# Autodesk Inventor assembly: towerbottom2.2
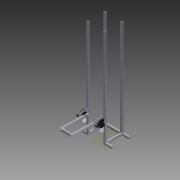
[picture p0: Inventor's stored thumbnail of the model, 180x180]
Saved by Autodesk Inventor 2011 SP1 (Build 150282100, 282)
## iProperties
Created: 2012-01-19
Part Number: towerbottom2.2
Document SubType Name: Assembly
Designer: Christopher
Author: Christopher
## Documents named in this file (12)
- C:\Users\Christopher\Documents\Christopher\FIRST\Inventor files\2012\tower bottom second design\towerbottom2.2.iam
- C:\Users\Christopher\Documents\Christopher\FIRST\Inventor files\2012\tower first design\towertallbackthing.ipt
- C:\Users\Christopher\Documents\Christopher\FIRST\Inventor files\2012\tower bottom second design\tower horizontal brace 17.5in.ipt
- C:\Users\Christopher\Documents\Christopher\FIRST\Inventor files\2012\tower bottom second design\towermiddle8inbrace.ipt
- C:\Users\Christopher\Documents\Christopher\FIRST\Inventor files\2012\tower bottom second design\towerside4.5inbrace.ipt
- C:\Users\Christopher\Documents\Christopher\FIRST\Inventor files\2011\Kit of Parts\motors\Motors_Denso_262100-3030.ipt
- C:\Users\Christopher\Documents\Christopher\FIRST\Inventor files\2011\Kit of Parts\motors\Motors_Denso_262100-3040.ipt
- C:\Users\Christopher\Documents\Christopher\FIRST\Inventor files\2012\tower bottom second design\window motor plate.ipt
- C:\Users\Christopher\Documents\Christopher\FIRST\Inventor files\2012\tower bottom second design\ramp1.ipt
- C:\Users\Christopher\Documents\Christopher\FIRST\Inventor files\2011\Kit of Parts\motors\Motors_Pelham Plastics_Denso-6.ipt
- C:\Users\Christopher\Documents\Christopher\FIRST\Inventor files\2012\tower bottom second design\bambar 12 in.ipt
- C:\Users\Christopher\Documents\Christopher\FIRST\Inventor files\2012\tower bottom second design\bambar 8.5 inch.ipt
## Components (19 placed, 11 different names)
1. towertallbackthing:1 — Mate:10, Flush:17, Flush:18, Flush:20, Mate:22
2. towertallbackthing:2 — Mate:9, Flush:21, Flush:22, Mate:21, Flush:27
3. towertallbackthing:3 — Mate:5, Flush:8, Flush:9
4. towertallbackthing:4 — Mate:6, Flush:10, Flush:11
5. tower horizontal brace 17.5in:2 — Mate:2, Flush:3, Flush:4, Mate:5, Flush:8, Flush:9, Mate:6, Flush:10, Flush:11, Flush:12, Mate:7, Flush:13, Mate:12, Flush:19
6. towermiddle8inbrace:1 — Mate:2, Flush:3, Flush:4, Mate:11, Flush:15, Flush:16, Flush:18, Mate:13
7. towermiddle8inbrace:2 — Flush:12, Mate:7, Flush:13, Mate:8, Flush:14, Mate:18, Flush:27
8. towerside4.5inbrace:1 — Mate:10, Mate:11, Flush:15, Flush:16, Flush:17, Mate:15
9. towerside4.5inbrace:2 — Mate:8, Flush:14, Mate:9, Mate:17, Flush:22
10. Motors_Denso_262100-3030:1 — Insert:1, Insert:4
11. Motors_Denso_262100-3040:1 — Insert:2, Insert:3
12. window motor plate:1 — Insert:1, Mate:15, Flush:20, Mate:22
13. window motor plate:2 — Mate:17, Flush:21, Insert:2, Mate:18, Mate:21
14. ramp1:1 — Mate:12, Flush:19, Mate:13
15. Motors_Pelham Plastics_Denso-6:1 — Insert:3, Insert:5, Insert:6
16. Motors_Pelham Plastics_Denso-6:2 — Insert:4
17. bambar 12 in:1 — Flush:23, Mate:19, Flush:24
18. bambar 12 in:2 — Mate:20, Flush:25, Flush:26, Insert:5, Insert:6
19. bambar 8.5 inch:1 — Flush:23, Mate:19, Flush:24, Mate:20, Flush:25, Flush:26
## Relationships (45: Flush 22, Mate 17, Insert 6)
- Mate:2: tower horizontal brace 17.5in:2 ↔ towermiddle8inbrace:1
- Flush:3: tower horizontal brace 17.5in:2 ↔ towermiddle8inbrace:1
- Flush:4 (-88.9 mm): tower horizontal brace 17.5in:2 ↔ towermiddle8inbrace:1
- Mate:5: towertallbackthing:3 ↔ tower horizontal brace 17.5in:2
- Flush:8: towertallbackthing:3 ↔ tower horizontal brace 17.5in:2
- Flush:9 (88.9 mm): towertallbackthing:3 ↔ tower horizontal brace 17.5in:2
- Mate:6: towertallbackthing:4 ↔ tower horizontal brace 17.5in:2
- Flush:10: towertallbackthing:4 ↔ tower horizontal brace 17.5in:2
- Flush:11 (88.9 mm): towertallbackthing:4 ↔ tower horizontal brace 17.5in:2
- Flush:12: tower horizontal brace 17.5in:2 ↔ towermiddle8inbrace:2
- Mate:7: tower horizontal brace 17.5in:2 ↔ towermiddle8inbrace:2
- Flush:13 (-88.9 mm): tower horizontal brace 17.5in:2 ↔ towermiddle8inbrace:2
- Mate:8: towermiddle8inbrace:2 ↔ towerside4.5inbrace:2
- Flush:14: towermiddle8inbrace:2 ↔ towerside4.5inbrace:2
- Mate:9: towertallbackthing:2 ↔ towerside4.5inbrace:2
- Mate:10: towertallbackthing:1 ↔ towerside4.5inbrace:1
- Mate:11: towermiddle8inbrace:1 ↔ towerside4.5inbrace:1
- Flush:15: towermiddle8inbrace:1 ↔ towerside4.5inbrace:1
- Flush:16: towermiddle8inbrace:1 ↔ towerside4.5inbrace:1
- Flush:17: towertallbackthing:1 ↔ towerside4.5inbrace:1
- Flush:18: towertallbackthing:1 ↔ towermiddle8inbrace:1
- Insert:1: Motors_Denso_262100-3030:1 ↔ window motor plate:1
- Mate:12: tower horizontal brace 17.5in:2 ↔ ramp1:1
- Flush:19: tower horizontal brace 17.5in:2 ↔ ramp1:1
- Mate:13: towermiddle8inbrace:1 ↔ ramp1:1
- Mate:15 (203.2 mm): towerside4.5inbrace:1 ↔ window motor plate:1
- Flush:20: towertallbackthing:1 ↔ window motor plate:1
- Mate:17 (203.2 mm): towerside4.5inbrace:2 ↔ window motor plate:2
- Flush:21: towertallbackthing:2 ↔ window motor plate:2
- Flush:22: towertallbackthing:2 ↔ towerside4.5inbrace:2
- Insert:2: Motors_Denso_262100-3040:1 ↔ window motor plate:2
- Mate:18 (203.2 mm): towermiddle8inbrace:2 ↔ window motor plate:2
- Insert:3: Motors_Denso_262100-3040:1 ↔ Motors_Pelham Plastics_Denso-6:1
- Insert:4: Motors_Denso_262100-3030:1 ↔ Motors_Pelham Plastics_Denso-6:2
- Flush:23: bambar 12 in:1 ↔ bambar 8.5 inch:1
- Mate:19: bambar 12 in:1 ↔ bambar 8.5 inch:1
- Flush:24: bambar 12 in:1 ↔ bambar 8.5 inch:1
- Mate:20: bambar 12 in:2 ↔ bambar 8.5 inch:1
- Flush:25: bambar 12 in:2 ↔ bambar 8.5 inch:1
- Flush:26: bambar 12 in:2 ↔ bambar 8.5 inch:1
- Insert:5: Motors_Pelham Plastics_Denso-6:1 ↔ bambar 12 in:2
- Insert:6: Motors_Pelham Plastics_Denso-6:1 ↔ bambar 12 in:2
- Mate:21: towertallbackthing:2 ↔ window motor plate:2
- Flush:27: towertallbackthing:2 ↔ towermiddle8inbrace:2
- Mate:22: towertallbackthing:1 ↔ window motor plate:1
